# Autodesk Inventor assembly: ServoAssembly
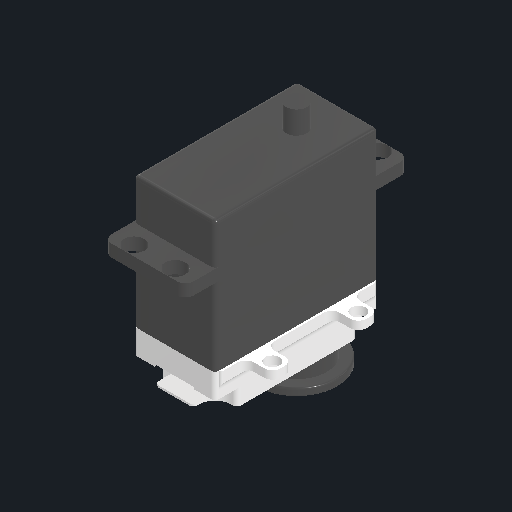
[picture p0: Inventor's stored thumbnail of the model, 512x512]
Saved by Autodesk Inventor 2026.2 (Build 302298010, 298A)
## iProperties
Created: 2026-02-18
Part Number: ServoAssembly
Document SubType Name: Assembly
Designer: Liam
Author: Liam
## Documents named in this file (4)
- C:\Users\Liam\OneDrive\Documents\Inventor\Hexapod\V2\ServoAssembly.iam
- C:\Users\Liam\OneDrive\Documents\Inventor\Hexapod\V2\Servo40KgNoBottom.ipt
- C:\Users\Liam\OneDrive\Documents\Inventor\Hexapod\V2\AxleCap.ipt
- C:\Users\Liam\OneDrive\Documents\Inventor\Hexapod\V2\ServoCase10mmTopHole.ipt
## Components (3 placed, 3 different names)
1. Servo40KgNoBottom:1 — Rigid:3
2. AxleCap:1 — Rigid:2
3. ServoCase10mmTopHole:1 — Rigid:2, Rigid:3
## Relationships (2: WeldJoint 2)
- Rigid:2 [WeldJoint]: AxleCap:1 ↔ ServoCase10mmTopHole:1
- Rigid:3 [WeldJoint]: Servo40KgNoBottom:1 ↔ ServoCase10mmTopHole:1
